# Autodesk Inventor assembly: Glider
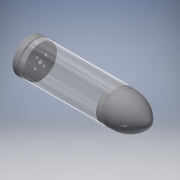
[picture p0: Inventor's stored thumbnail of the model, 180x180]
Saved by Autodesk Inventor 2018.3 (Build 223284000, 284)
## iProperties
Created: 2019-03-19
Part Number: Glider
Document SubType Name: Assembly
Designer: Mario
Author: Mario
## Documents named in this file (7)
- C:\Users\Mario\Documents\Inventor\Underwater glider\Glider.iam
- C:\Users\Mario\Documents\Inventor\Underwater glider\Tubo.ipt
- C:\Users\Mario\Documents\Inventor\Underwater glider\Tapon 2.ipt
- C:\Users\Mario\Documents\Inventor\Underwater glider\Tapon 1.ipt
- C:\Users\Mario\Documents\Inventor\Underwater glider\Cabeza.ipt
- C:\Users\Mario\Documents\Inventor\Underwater glider\Tapon 1_Cabeza.ipt
- C:\Users\Mario\Documents\Inventor\Underwater glider\Cabeza_diseño2.ipt
## Components (7 placed, 6 different names)
1. Tubo:1 — Cylindrical:1, Cylindrical:2, Mate:1
2. Tapon 1:1 — Rotational:1, Mate:1
3. Tapon 2:1 — Cylindrical:2, Rotational:2
4. Tapon 2:2 — Cylindrical:1, Rotational:1
5. Tapon 1_Cabeza:1 — Rotational:2, Rotational:4
6. Cabeza:1
7. Cabeza_diseño2:1 — Rotational:4
## Relationships (6: RevoluteJoint 3, CylindricalJoint 2, Mate 1)
- Cylindrical:1: Tubo:1 ↔ Tapon 2:2
- Rotational:1 [RevoluteJoint]: Tapon 1:1 ↔ Tapon 2:2
- Cylindrical:2: Tubo:1 ↔ Tapon 2:1
- Rotational:2 [RevoluteJoint]: Tapon 2:1 ↔ Tapon 1_Cabeza:1
- Mate:1: Tubo:1 ↔ Tapon 1:1
- Rotational:4 [RevoluteJoint]: Tapon 1_Cabeza:1 ↔ Cabeza_diseño2:1
